# Autodesk Inventor assembly: Assembly
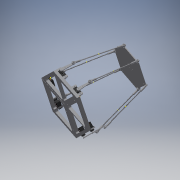
[picture p0: Inventor's stored thumbnail of the model, 180x180]
Saved by Autodesk Inventor 2019 (Build 230136000, 136)
## iProperties
Created: 2019-09-23
Part Number: Assembly
Document SubType Name: Assembly
Designer: Jorian Brusind
Author: Jorian Brusind
## Documents named in this file (8)
- C:\Users\Jorian Brusind\Documents\GitHub\PersonalProjects\RPI Stellar Photography\Inventor Files\Test Stewart Platform\Assembly.iam
- C:\Users\Jorian Brusind\Documents\GitHub\PersonalProjects\RPI Stellar Photography\Inventor Files\Test Stewart Platform\Hex_Servo_Base.ipt
- C:\Users\Jorian Brusind\Documents\GitHub\PersonalProjects\RPI Stellar Photography\Inventor Files\Test Stewart Platform\Servo\SG90.ipt
- C:\Users\Jorian Brusind\Documents\GitHub\PersonalProjects\RPI Stellar Photography\Inventor Files\Test Stewart Platform\Servo\SG90 - Micro Servo 9g - Tower Pro.2.ipt
- C:\Users\Jorian Brusind\Documents\GitHub\PersonalProjects\RPI Stellar Photography\Inventor Files\Test Stewart Platform\Servo_Arm.ipt
- C:\Users\Jorian Brusind\Documents\GitHub\PersonalProjects\RPI Stellar Photography\Inventor Files\Test Stewart Platform\Hex_Servo_Top.ipt
- C:\Users\Jorian Brusind\Documents\GitHub\PersonalProjects\RPI Stellar Photography\Inventor Files\Test Stewart Platform\Arm.iam
- C:\Users\Jorian Brusind\Documents\GitHub\PersonalProjects\RPI Stellar Photography\Inventor Files\raspberry-pi-camera-module-v2-1.snapshot.3\RspCameraMia.iam
## Components (29 placed, 7 different names)
1. Hex_Servo_Base:1 — Mate:1, Mate:2, Mate:3, Mate:18, Mate:19, Mate:20, Mate:21, Mate:22, Mate:23
2. Hex_Servo_Base:2 — Mate:1, Mate:2, Mate:3, Flush:1, Mate:12, Mate:13, Mate:14, Mate:15, Mate:16, Mate:17, Mate:62, Mate:63
3. Hex_Servo_Base:3 — Flush:1, Mate:6, Mate:7, Mate:8, Mate:9, Mate:10, Mate:11, Mate:62, Mate:63
4. SG90:1 — Mate:9, Mate:10, Mate:11, Mate:32, Mate:33
5. SG90:2 — Mate:6, Mate:7, Mate:8, Mate:34, Mate:35
6. SG90:3 — Mate:21, Mate:22, Mate:23, Mate:26, Mate:27
7. SG90:4 — Mate:18, Mate:19, Mate:20, Mate:24, Mate:25
8. SG90:5 — Mate:15, Mate:16, Mate:17, Mate:28, Mate:29
9. SG90:6 — Mate:12, Mate:13, Mate:14, Mate:30, Mate:31
10. SG90 - Micro Servo 9g - Tower Pro.2:1 — Mate:26, Mate:27, Mate:41, Mate:42, Mate:43
11. SG90 - Micro Servo 9g - Tower Pro.2:2 — Mate:28, Mate:29, Mate:53, Mate:54, Mate:55
12. SG90 - Micro Servo 9g - Tower Pro.2:3 — Mate:30, Mate:31, Mate:50, Mate:51, Mate:52
13. SG90 - Micro Servo 9g - Tower Pro.2:4 — Mate:24, Mate:25, Mate:38, Mate:39, Mate:40
14. SG90 - Micro Servo 9g - Tower Pro.2:5 — Mate:32, Mate:33, Mate:47, Mate:48, Mate:49
15. SG90 - Micro Servo 9g - Tower Pro.2:6 — Mate:34, Mate:35, Mate:44, Mate:45, Mate:46
16. Servo_Arm:1 — Mate:38, Mate:39, Mate:40, Ball:3
17. Servo_Arm:2 — Mate:50, Mate:51, Mate:52, Ball:7
18. Servo_Arm:3 — Mate:41, Mate:42, Mate:43, Ball:1
19. Servo_Arm:4 — Mate:53, Mate:54, Mate:55, Ball:5
20. Servo_Arm:5 — Mate:44, Mate:45, Mate:46, Ball:9
21. Servo_Arm:6 — Mate:47, Mate:48, Mate:49, Ball:11
22. Hex_Servo_Top:1 — Ball:2, Ball:4, Ball:6, Ball:8, Ball:10, Ball:12, Mate:64, Mate:65, Mate:66
23. Arm:2 [sub-assembly] — Ball:7, Ball:8
24. Arm:3 [sub-assembly] — Ball:3, Ball:4
25. Arm:4 [sub-assembly] — Ball:1, Ball:2
26. Arm:5 [sub-assembly] — Ball:5, Ball:6
27. Arm:6 [sub-assembly] — Ball:9, Ball:10
28. Arm:7 [sub-assembly] — Ball:11, Ball:12
29. RspCameraMia:1 [sub-assembly] — Mate:64, Mate:65, Mate:66
## Relationships (69: Mate 56, BallJoint 12, Flush 1)
- Mate:1 (0.5 mm): Hex_Servo_Base:1 ↔ Hex_Servo_Base:2
- Mate:2: Hex_Servo_Base:1 ↔ Hex_Servo_Base:2
- Mate:3 (0.5 mm): Hex_Servo_Base:1 ↔ Hex_Servo_Base:2
- Flush:1: Hex_Servo_Base:2 ↔ Hex_Servo_Base:3
- Mate:6: Hex_Servo_Base:3 ↔ SG90:2
- Mate:7: Hex_Servo_Base:3 ↔ SG90:2
- Mate:8: Hex_Servo_Base:3 ↔ SG90:2
- Mate:9: Hex_Servo_Base:3 ↔ SG90:1
- Mate:10: Hex_Servo_Base:3 ↔ SG90:1
- Mate:11: Hex_Servo_Base:3 ↔ SG90:1
- Mate:12: Hex_Servo_Base:2 ↔ SG90:6
- Mate:13: Hex_Servo_Base:2 ↔ SG90:6
- Mate:14: Hex_Servo_Base:2 ↔ SG90:6
- Mate:15: Hex_Servo_Base:2 ↔ SG90:5
- Mate:16: Hex_Servo_Base:2 ↔ SG90:5
- Mate:17: Hex_Servo_Base:2 ↔ SG90:5
- Mate:18: Hex_Servo_Base:1 ↔ SG90:4
- Mate:19: Hex_Servo_Base:1 ↔ SG90:4
- Mate:20: Hex_Servo_Base:1 ↔ SG90:4
- Mate:21: Hex_Servo_Base:1 ↔ SG90:3
- Mate:22: Hex_Servo_Base:1 ↔ SG90:3
- Mate:23: Hex_Servo_Base:1 ↔ SG90:3
- Mate:24: SG90:4 ↔ SG90 - Micro Servo 9g - Tower Pro.2:4
- Mate:25: SG90:4 ↔ SG90 - Micro Servo 9g - Tower Pro.2:4
- Mate:26: SG90:3 ↔ SG90 - Micro Servo 9g - Tower Pro.2:1
- Mate:27: SG90:3 ↔ SG90 - Micro Servo 9g - Tower Pro.2:1
- Mate:28: SG90:5 ↔ SG90 - Micro Servo 9g - Tower Pro.2:2
- Mate:29: SG90:5 ↔ SG90 - Micro Servo 9g - Tower Pro.2:2
- Mate:30: SG90:6 ↔ SG90 - Micro Servo 9g - Tower Pro.2:3
- Mate:31: SG90:6 ↔ SG90 - Micro Servo 9g - Tower Pro.2:3
- Mate:32: SG90:1 ↔ SG90 - Micro Servo 9g - Tower Pro.2:5
- Mate:33: SG90:1 ↔ SG90 - Micro Servo 9g - Tower Pro.2:5
- Mate:34: SG90:2 ↔ SG90 - Micro Servo 9g - Tower Pro.2:6
- Mate:35: SG90:2 ↔ SG90 - Micro Servo 9g - Tower Pro.2:6
- Mate:38: SG90 - Micro Servo 9g - Tower Pro.2:4 ↔ Servo_Arm:1
- Mate:39: SG90 - Micro Servo 9g - Tower Pro.2:4 ↔ Servo_Arm:1
- Mate:40: SG90 - Micro Servo 9g - Tower Pro.2:4 ↔ Servo_Arm:1
- Mate:41: SG90 - Micro Servo 9g - Tower Pro.2:1 ↔ Servo_Arm:3
- Mate:42: SG90 - Micro Servo 9g - Tower Pro.2:1 ↔ Servo_Arm:3
- Mate:43: SG90 - Micro Servo 9g - Tower Pro.2:1 ↔ Servo_Arm:3
- Mate:44: SG90 - Micro Servo 9g - Tower Pro.2:6 ↔ Servo_Arm:5
- Mate:45: SG90 - Micro Servo 9g - Tower Pro.2:6 ↔ Servo_Arm:5
- Mate:46: SG90 - Micro Servo 9g - Tower Pro.2:6 ↔ Servo_Arm:5
- Mate:47: SG90 - Micro Servo 9g - Tower Pro.2:5 ↔ Servo_Arm:6
- Mate:48: SG90 - Micro Servo 9g - Tower Pro.2:5 ↔ Servo_Arm:6
- Mate:49: SG90 - Micro Servo 9g - Tower Pro.2:5 ↔ Servo_Arm:6
- Mate:50: SG90 - Micro Servo 9g - Tower Pro.2:3 ↔ Servo_Arm:2
- Mate:51: SG90 - Micro Servo 9g - Tower Pro.2:3 ↔ Servo_Arm:2
- Mate:52: SG90 - Micro Servo 9g - Tower Pro.2:3 ↔ Servo_Arm:2
- Mate:53: SG90 - Micro Servo 9g - Tower Pro.2:2 ↔ Servo_Arm:4
- Mate:54: SG90 - Micro Servo 9g - Tower Pro.2:2 ↔ Servo_Arm:4
- Mate:55: SG90 - Micro Servo 9g - Tower Pro.2:2 ↔ Servo_Arm:4
- Mate:62 (0.4 mm): Hex_Servo_Base:2 ↔ Hex_Servo_Base:3
- Mate:63 (0.5 mm): Hex_Servo_Base:2 ↔ Hex_Servo_Base:3
- Ball:1: Servo_Arm:3 ↔ Arm:4
- Ball:2: Hex_Servo_Top:1 ↔ Arm:4
- Ball:3: Servo_Arm:1 ↔ Arm:3
- Ball:4: Hex_Servo_Top:1 ↔ Arm:3
- Ball:5: Servo_Arm:4 ↔ Arm:5
- Ball:6: Hex_Servo_Top:1 ↔ Arm:5
- Ball:7: Servo_Arm:2 ↔ Arm:2
- Ball:8: Hex_Servo_Top:1 ↔ Arm:2
- Ball:9: Servo_Arm:5 ↔ Arm:6
- Ball:10: Hex_Servo_Top:1 ↔ Arm:6
- Ball:11: Servo_Arm:6 ↔ Arm:7
- Ball:12: Hex_Servo_Top:1 ↔ Arm:7
- Mate:64: Hex_Servo_Top:1 ↔ RspCameraMia:1
- Mate:65: Hex_Servo_Top:1 ↔ RspCameraMia:1
- Mate:66: Hex_Servo_Top:1 ↔ RspCameraMia:1
